# Autodesk Inventor assembly: Assembly Rack
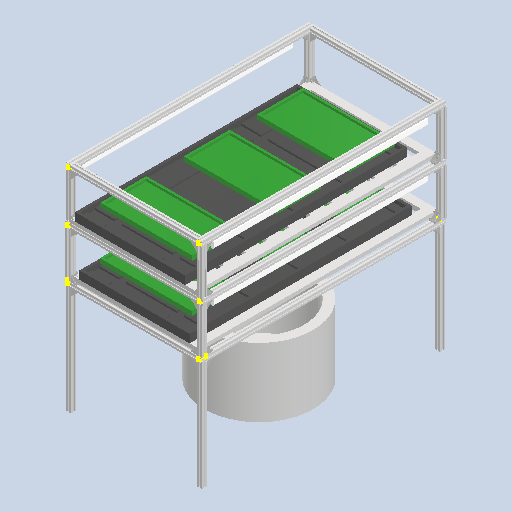
[picture p0: Inventor's stored thumbnail of the model, 512x512]
Saved by Autodesk Inventor 2025 (Build 290162000, 162)
## iProperties
Created: 2024-06-18
Part Number: Assembly Rack
Document SubType Name: Assembly
Designer: Isaac
Author: Isaac
## Documents named in this file (11)
- C:\Users\User\OneDrive\Documents\FYP\Inventor_Designs\Rack\Assembly Rack.iam
- C:\Users\User\OneDrive\Documents\FYP\Inventor_Designs\Rack\Metal_Profile 135cm.ipt
- C:\Users\User\OneDrive\Documents\FYP\Inventor_Designs\Rack\Metal_Profile 70cm.ipt
- C:\Users\User\OneDrive\Documents\FYP\Inventor_Designs\Rack\Metal Profile 25cm.ipt
- C:\Users\User\OneDrive\Documents\FYP\Inventor_Designs\Rack\Metal_Profile 60cm.ipt
- C:\Users\User\OneDrive\Documents\FYP\Inventor_Designs\Rack\Light tube 118.4cm.ipt
- C:\Users\User\OneDrive\Documents\FYP\Inventor_Designs\L Bracket\L Angle Bracket 30x30.ipt
- C:\Users\User\OneDrive\Documents\FYP\Inventor_Designs\Rack\Part3.ipt
- C:\Users\User\OneDrive\Documents\FYP\Inventor_Designs\Rack\Tub.ipt
- C:\Users\User\OneDrive\Documents\FYP\Inventor_Designs\Rack\flood tray.ipt
- C:\Users\User\OneDrive\Documents\FYP\Inventor_Designs\Platform\Potting Tray.ipt
## Components (79 placed, 10 different names)
1. Metal_Profile 70cm:1 — Mate:1, Mate:2, Mate:3, Mate:12, Mate:14, Mate:52, Mate:64, Mate:65, Mate:66, Mate:69
2. Metal_Profile 70cm:2 — Mate:4, Mate:5, Mate:13, Mate:15, Mate:54, Mate:75, Mate:123
3. Metal_Profile 135cm:2 — Mate:5, Mate:6, Mate:7, Mate:8, Mate:43, Mate:84, Mate:90, Mate:91, Mate:118
4. Metal_Profile 135cm:1 — Mate:1, Mate:2, Mate:3, Mate:4, Mate:9, Mate:10, Mate:11, Mate:41, Mate:86, Mate:99, Mate:106, Mate:120, Mate:124
5. Metal Profile 25cm:1 — Mate:6, Mate:25, Mate:26, Mate:62, Mate:70, Mate:89, Mate:100
6. Metal Profile 25cm:2 — Mate:7, Mate:8, Mate:27, Mate:63, Mate:72, Mate:83, Mate:113
7. Metal Profile 25cm:3 — Mate:9, Mate:29, Mate:49, Mate:59, Mate:98, Mate:102
8. Metal Profile 25cm:4 — Mate:10, Mate:11, Mate:28, Mate:55, Mate:58, Mate:85, Mate:115
9. Metal Profile 25cm:6 — Mate:12, Mate:16, Mate:17, Mate:44, Mate:51, Mate:96, Mate:105
10. Metal Profile 25cm:7 — Mate:13, Mate:18, Mate:47, Mate:53, Mate:80, Mate:119
11. Metal Profile 25cm:8 — Mate:14, Mate:19, Mate:60, Mate:67, Mate:68, Mate:87, Mate:104
12. Metal Profile 25cm:9 — Mate:15, Mate:20, Mate:61, Mate:74, Mate:82, Mate:117
13. Metal_Profile 135cm:3 — Mate:16, Mate:17, Mate:18, Mate:23, Mate:24, Mate:40, Mate:81, Mate:97
14. Metal_Profile 135cm:4 — Mate:19, Mate:20, Mate:21, Mate:22, Mate:42, Mate:88
15. Metal_Profile 70cm:3 — Mate:21, Mate:22, Mate:45, Mate:46
16. Metal_Profile 70cm:4 — Mate:23, Mate:24, Mate:48
17. Metal_Profile 135cm:5 — Mate:25, Mate:26, Mate:27, Mate:30, Mate:31, Mate:35, Mate:36, Mate:37, Mate:38, Mate:93, Mate:101, Mate:108, Mate:114
18. Metal_Profile 135cm:6 — Mate:28, Mate:29, Mate:32, Mate:33, Mate:34, Mate:39, Mate:95, Mate:103, Mate:110, Mate:116
19. Metal_Profile 70cm:5 — Mate:32, Mate:50, Mate:57, Mate:71, Mate:77, Mate:125, Mate:126
20. Metal_Profile 70cm:6 — Mate:30, Mate:31, Mate:73, Mate:79, Mate:112
21. Metal_Profile 60cm:1 — Mate:39, Mate:56, Mate:94
22. Metal_Profile 60cm:2 — Mate:35, Mate:36, Mate:78, Mate:107
23. Metal_Profile 60cm:3 — Mate:33, Mate:34, Mate:109, Mate:111
24. Metal_Profile 60cm:4 — Mate:37, Mate:38, Mate:76, Mate:92
25. Light tube 118.4cm:1 — Mate:40
26. Light tube 118.4cm:2 — Mate:42
27. Light tube 118.4cm:3 — Mate:41
28. Light tube 118.4cm:4 — Mate:43, Mate:91
29. L Angle Bracket 30x30:5 — Mate:47, Mate:48
30. L Angle Bracket 30x30:6 — Mate:44, Mate:45, Mate:46
31. L Angle Bracket 30x30:7 — Mate:49, Mate:50, Mate:125
32. L Angle Bracket 30x30:8 — Mate:51, Mate:52
33. L Angle Bracket 30x30:9 — Mate:53, Mate:54
34. L Angle Bracket 30x30:10 — Mate:55
35. L Angle Bracket 30x30:11 — Mate:56, Mate:57
36. L Angle Bracket 30x30:12 — Mate:59
37. L Angle Bracket 30x30:13 — Mate:58
38. L Angle Bracket 30x30:14 — Mate:60, Mate:67
39. L Angle Bracket 30x30:15 — Mate:61
40. L Angle Bracket 30x30:16 — Mate:62, Mate:64, Mate:65, Mate:66
41. L Angle Bracket 30x30:17 — Mate:63
42. L Angle Bracket 30x30:18 — Mate:70, Mate:71
43. L Angle Bracket 30x30:19 — Mate:68, Mate:69
44. L Angle Bracket 30x30:20 — Mate:74, Mate:75
45. L Angle Bracket 30x30:21 — Mate:72, Mate:73
46. L Angle Bracket 30x30:22 — Mate:76, Mate:77
47. L Angle Bracket 30x30:24 — Mate:78, Mate:79
48. L Angle Bracket 30x30:25 — Mate:82
49. L Angle Bracket 30x30:26 — Mate:80, Mate:81
50. L Angle Bracket 30x30:27 — Mate:83, Mate:84
51. L Angle Bracket 30x30:28 — Mate:85, Mate:86
52. L Angle Bracket 30x30:29 — Mate:87, Mate:88
53. L Angle Bracket 30x30:30 — Mate:89, Mate:90
54. L Angle Bracket 30x30:31 — Mate:92, Mate:93
55. L Angle Bracket 30x30:32 — Mate:94, Mate:95
56. L Angle Bracket 30x30:33 — Mate:96, Mate:97
57. L Angle Bracket 30x30:34 — Mate:98, Mate:99
58. L Angle Bracket 30x30:35 — Mate:104
59. L Angle Bracket 30x30:36 — Mate:105, Mate:106
60. L Angle Bracket 30x30:37 — Mate:100, Mate:101
61. L Angle Bracket 30x30:38 — Mate:102, Mate:103
62. L Angle Bracket 30x30:39 — Mate:109, Mate:110
63. L Angle Bracket 30x30:40 — Mate:107, Mate:108
64. L Angle Bracket 30x30:41 — Mate:111, Mate:112
65. L Angle Bracket 30x30:42 — Mate:117, Mate:118
66. L Angle Bracket 30x30:43 — Mate:119, Mate:120
67. L Angle Bracket 30x30:44 — Mate:113, Mate:114
68. L Angle Bracket 30x30:45 — Mate:115, Mate:116
69. Part3:1 — Mate:123, Mate:124, Mate:127
70. Part3:2 — Mate:126, Mate:128
71. Tub:1
72. flood tray:1 — Mate:127
73. flood tray:2 — Mate:128
74. Potting Tray:1
75. Potting Tray:2
76. Potting Tray:3
77. Potting Tray:4
78. Potting Tray:5
79. Potting Tray:6
## Relationships (126: Mate 126)
- Mate:1: Metal_Profile 70cm:1 ↔ Metal_Profile 135cm:1
- Mate:2: Metal_Profile 70cm:1 ↔ Metal_Profile 135cm:1
- Mate:3: Metal_Profile 70cm:1 ↔ Metal_Profile 135cm:1
- Mate:4: Metal_Profile 70cm:2 ↔ Metal_Profile 135cm:1
- Mate:5: Metal_Profile 70cm:2 ↔ Metal_Profile 135cm:2
- Mate:6: Metal_Profile 135cm:2 ↔ Metal Profile 25cm:1
- Mate:7: Metal_Profile 135cm:2 ↔ Metal Profile 25cm:2
- Mate:8: Metal_Profile 135cm:2 ↔ Metal Profile 25cm:2
- Mate:9: Metal_Profile 135cm:1 ↔ Metal Profile 25cm:3
- Mate:10: Metal_Profile 135cm:1 ↔ Metal Profile 25cm:4
- Mate:11: Metal_Profile 135cm:1 ↔ Metal Profile 25cm:4
- Mate:12: Metal_Profile 70cm:1 ↔ Metal Profile 25cm:6
- Mate:13: Metal_Profile 70cm:2 ↔ Metal Profile 25cm:7
- Mate:14: Metal_Profile 70cm:1 ↔ Metal Profile 25cm:8
- Mate:15: Metal_Profile 70cm:2 ↔ Metal Profile 25cm:9
- Mate:16: Metal Profile 25cm:6 ↔ Metal_Profile 135cm:3
- Mate:17: Metal Profile 25cm:6 ↔ Metal_Profile 135cm:3
- Mate:18: Metal Profile 25cm:7 ↔ Metal_Profile 135cm:3
- Mate:19: Metal Profile 25cm:8 ↔ Metal_Profile 135cm:4
- Mate:20: Metal Profile 25cm:9 ↔ Metal_Profile 135cm:4
- Mate:21: Metal_Profile 135cm:4 ↔ Metal_Profile 70cm:3
- Mate:22: Metal_Profile 135cm:4 ↔ Metal_Profile 70cm:3
- Mate:23: Metal_Profile 135cm:3 ↔ Metal_Profile 70cm:4
- Mate:24: Metal_Profile 135cm:3 ↔ Metal_Profile 70cm:4
- Mate:25: Metal Profile 25cm:1 ↔ Metal_Profile 135cm:5
- Mate:26: Metal Profile 25cm:1 ↔ Metal_Profile 135cm:5
- Mate:27: Metal Profile 25cm:2 ↔ Metal_Profile 135cm:5
- Mate:28: Metal Profile 25cm:4 ↔ Metal_Profile 135cm:6
- Mate:29: Metal Profile 25cm:3 ↔ Metal_Profile 135cm:6
- Mate:30: Metal_Profile 135cm:5 ↔ Metal_Profile 70cm:6
- Mate:31: Metal_Profile 135cm:5 ↔ Metal_Profile 70cm:6
- Mate:32: Metal_Profile 135cm:6 ↔ Metal_Profile 70cm:5
- Mate:33: Metal_Profile 135cm:6 ↔ Metal_Profile 60cm:3
- Mate:34: Metal_Profile 135cm:6 ↔ Metal_Profile 60cm:3
- Mate:35: Metal_Profile 135cm:5 ↔ Metal_Profile 60cm:2
- Mate:36: Metal_Profile 135cm:5 ↔ Metal_Profile 60cm:2
- Mate:37: Metal_Profile 135cm:5 ↔ Metal_Profile 60cm:4
- Mate:38: Metal_Profile 135cm:5 ↔ Metal_Profile 60cm:4
- Mate:39: Metal_Profile 135cm:6 ↔ Metal_Profile 60cm:1
- Mate:40: Metal_Profile 135cm:3 ↔ Light tube 118.4cm:1
- Mate:41: Metal_Profile 135cm:1 ↔ Light tube 118.4cm:3
- Mate:42: Metal_Profile 135cm:4 ↔ Light tube 118.4cm:2
- Mate:43: Metal_Profile 135cm:2 ↔ Light tube 118.4cm:4
- Mate:44: Metal Profile 25cm:6 ↔ L Angle Bracket 30x30:6
- Mate:45: Metal_Profile 70cm:3 ↔ L Angle Bracket 30x30:6
- Mate:46: Metal_Profile 70cm:3 ↔ L Angle Bracket 30x30:6
- Mate:47: Metal Profile 25cm:7 ↔ L Angle Bracket 30x30:5
- Mate:48: Metal_Profile 70cm:4 ↔ L Angle Bracket 30x30:5
- Mate:49: Metal Profile 25cm:3 ↔ L Angle Bracket 30x30:7
- Mate:50: Metal_Profile 70cm:5 ↔ L Angle Bracket 30x30:7
- Mate:51: Metal Profile 25cm:6 ↔ L Angle Bracket 30x30:8
- Mate:52: Metal_Profile 70cm:1 ↔ L Angle Bracket 30x30:8
- Mate:53: Metal Profile 25cm:7 ↔ L Angle Bracket 30x30:9
- Mate:54: Metal_Profile 70cm:2 ↔ L Angle Bracket 30x30:9
- Mate:55: Metal Profile 25cm:4 ↔ L Angle Bracket 30x30:10
- Mate:56: Metal_Profile 60cm:1 ↔ L Angle Bracket 30x30:11
- Mate:57: Metal_Profile 70cm:5 ↔ L Angle Bracket 30x30:11
- Mate:58: Metal Profile 25cm:4 ↔ L Angle Bracket 30x30:13
- Mate:59: Metal Profile 25cm:3 ↔ L Angle Bracket 30x30:12
- Mate:60: Metal Profile 25cm:8 ↔ L Angle Bracket 30x30:14
- Mate:61: Metal Profile 25cm:9 ↔ L Angle Bracket 30x30:15
- Mate:62: Metal Profile 25cm:1 ↔ L Angle Bracket 30x30:16
- Mate:63: Metal Profile 25cm:2 ↔ L Angle Bracket 30x30:17
- Mate:64: Metal_Profile 70cm:1 ↔ L Angle Bracket 30x30:16
- Mate:65: Metal_Profile 70cm:1 ↔ L Angle Bracket 30x30:16
- Mate:66: Metal_Profile 70cm:1 ↔ L Angle Bracket 30x30:16
- Mate:67: Metal Profile 25cm:8 ↔ L Angle Bracket 30x30:14
- Mate:68: Metal Profile 25cm:8 ↔ L Angle Bracket 30x30:19
- Mate:69: Metal_Profile 70cm:1 ↔ L Angle Bracket 30x30:19
- Mate:70: Metal Profile 25cm:1 ↔ L Angle Bracket 30x30:18
- Mate:71: Metal_Profile 70cm:5 ↔ L Angle Bracket 30x30:18
- Mate:72: Metal Profile 25cm:2 ↔ L Angle Bracket 30x30:21
- Mate:73: Metal_Profile 70cm:6 ↔ L Angle Bracket 30x30:21
- Mate:74: Metal Profile 25cm:9 ↔ L Angle Bracket 30x30:20
- Mate:75: Metal_Profile 70cm:2 ↔ L Angle Bracket 30x30:20
- Mate:76: Metal_Profile 60cm:4 ↔ L Angle Bracket 30x30:22
- Mate:77: Metal_Profile 70cm:5 ↔ L Angle Bracket 30x30:22
- Mate:78: Metal_Profile 60cm:2 ↔ L Angle Bracket 30x30:24
- Mate:79: Metal_Profile 70cm:6 ↔ L Angle Bracket 30x30:24
- Mate:80: Metal Profile 25cm:7 ↔ L Angle Bracket 30x30:26
- Mate:81: Metal_Profile 135cm:3 ↔ L Angle Bracket 30x30:26
- Mate:82: Metal Profile 25cm:9 ↔ L Angle Bracket 30x30:25
- Mate:83: Metal Profile 25cm:2 ↔ L Angle Bracket 30x30:27
- Mate:84: Metal_Profile 135cm:2 ↔ L Angle Bracket 30x30:27
- Mate:85: Metal Profile 25cm:4 ↔ L Angle Bracket 30x30:28
- Mate:86: Metal_Profile 135cm:1 ↔ L Angle Bracket 30x30:28
- Mate:87: Metal Profile 25cm:8 ↔ L Angle Bracket 30x30:29
- Mate:88: Metal_Profile 135cm:4 ↔ L Angle Bracket 30x30:29
- Mate:89: Metal Profile 25cm:1 ↔ L Angle Bracket 30x30:30
- Mate:90: Metal_Profile 135cm:2 ↔ L Angle Bracket 30x30:30
- Mate:91: Metal_Profile 135cm:2 ↔ Light tube 118.4cm:4
- Mate:92: Metal_Profile 60cm:4 ↔ L Angle Bracket 30x30:31
- Mate:93: Metal_Profile 135cm:5 ↔ L Angle Bracket 30x30:31
- Mate:94: Metal_Profile 60cm:1 ↔ L Angle Bracket 30x30:32
- Mate:95: Metal_Profile 135cm:6 ↔ L Angle Bracket 30x30:32
- Mate:96: Metal Profile 25cm:6 ↔ L Angle Bracket 30x30:33
- Mate:97: Metal_Profile 135cm:3 ↔ L Angle Bracket 30x30:33
- Mate:98: Metal Profile 25cm:3 ↔ L Angle Bracket 30x30:34
- Mate:99: Metal_Profile 135cm:1 ↔ L Angle Bracket 30x30:34
- Mate:100: Metal Profile 25cm:1 ↔ L Angle Bracket 30x30:37
- Mate:101: Metal_Profile 135cm:5 ↔ L Angle Bracket 30x30:37
- Mate:102: Metal Profile 25cm:3 ↔ L Angle Bracket 30x30:38
- Mate:103: Metal_Profile 135cm:6 ↔ L Angle Bracket 30x30:38
- Mate:104: Metal Profile 25cm:8 ↔ L Angle Bracket 30x30:35
- Mate:105: Metal Profile 25cm:6 ↔ L Angle Bracket 30x30:36
- Mate:106: Metal_Profile 135cm:1 ↔ L Angle Bracket 30x30:36
- Mate:107: Metal_Profile 60cm:2 ↔ L Angle Bracket 30x30:40
- Mate:108: Metal_Profile 135cm:5 ↔ L Angle Bracket 30x30:40
- Mate:109: Metal_Profile 60cm:3 ↔ L Angle Bracket 30x30:39
- Mate:110: Metal_Profile 135cm:6 ↔ L Angle Bracket 30x30:39
- Mate:111: Metal_Profile 60cm:3 ↔ L Angle Bracket 30x30:41
- Mate:112: Metal_Profile 70cm:6 ↔ L Angle Bracket 30x30:41
- Mate:113: Metal Profile 25cm:2 ↔ L Angle Bracket 30x30:44
- Mate:114: Metal_Profile 135cm:5 ↔ L Angle Bracket 30x30:44
- Mate:115: Metal Profile 25cm:4 ↔ L Angle Bracket 30x30:45
- Mate:116: Metal_Profile 135cm:6 ↔ L Angle Bracket 30x30:45
- Mate:117: Metal Profile 25cm:9 ↔ L Angle Bracket 30x30:42
- Mate:118: Metal_Profile 135cm:2 ↔ L Angle Bracket 30x30:42
- Mate:119: Metal Profile 25cm:7 ↔ L Angle Bracket 30x30:43
- Mate:120: Metal_Profile 135cm:1 ↔ L Angle Bracket 30x30:43
- Mate:123: Metal_Profile 70cm:2 ↔ Part3:1
- Mate:124: Metal_Profile 135cm:1 ↔ Part3:1
- Mate:125: Metal_Profile 70cm:5 ↔ L Angle Bracket 30x30:7
- Mate:126: Metal_Profile 70cm:5 ↔ Part3:2
- Mate:127: Part3:1 ↔ flood tray:1
- Mate:128: Part3:2 ↔ flood tray:2
